# Autodesk Inventor assembly: Ensemble1
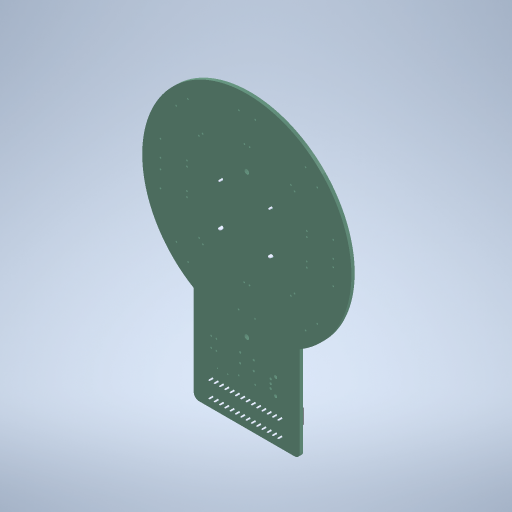
[picture p0: Inventor's stored thumbnail of the model, 512x512]
Saved by Autodesk Inventor 2024 (Build 280153000, 153)
## iProperties
Created: 2023-11-16
Part Number: Ensemble1
Document SubType Name: Assembly
Designer: digiacom
Author: digiacom
## Documents named in this file (5)
- D:\Projet\Perso\ATMegaSpin\Inventor\Ensemble1.iam
- D:\Projet\Perso\ATMegaSpin\3DModel\ATMegaSpin\ATMegaSpin.ipt
- D:\Projet\Perso\ATMegaSpin\3DModel\Parts\BS-7--3DModel-STEP-1\BS-7--3DModel-STEP-1.ipt
- D:\Projet\Perso\ATMegaSpin\3DModel\Parts\ED281DT\ED281DT.ipt
- D:\Projet\Perso\ATMegaSpin\3DModel\Parts\ATMEGA328P-PU\ATMEGA328P-PU.ipt
## Components (5 placed, 4 different names)
1. ATMegaSpin:1 — Placage:2, Placage:3, Placage:4, Placage:5
2. BS-7--3DModel-STEP-1:1 — Placage:2, Placage:3
3. BS-7--3DModel-STEP-1:2 — Placage:4, Placage:5
4. ED281DT:2
5. ATMEGA328P-PU:1
## Relationships (4: Mate 4)
- Placage:2 [Mate]: ATMegaSpin:1 ↔ BS-7--3DModel-STEP-1:1
- Placage:3 [Mate] (0.7 mm): ATMegaSpin:1 ↔ BS-7--3DModel-STEP-1:1
- Placage:4 [Mate]: ATMegaSpin:1 ↔ BS-7--3DModel-STEP-1:2
- Placage:5 [Mate] (-0.35 mm): ATMegaSpin:1 ↔ BS-7--3DModel-STEP-1:2
